# Autodesk Inventor assembly: FEM-Träger-Baugruppe1
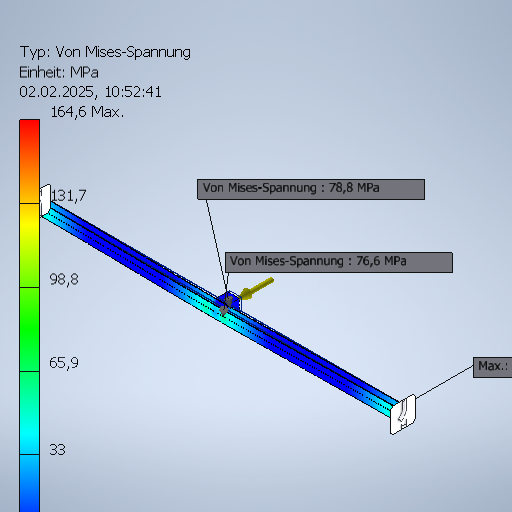
[picture p0: Inventor's stored thumbnail of the model, 512x512]
Saved by Autodesk Inventor 2025 (Build 290162010, 162A)
## iProperties
Created: 2025-02-02
Part Number: FEM-Träger-Baugruppe1
Document SubType Name: Assembly
Designer: Admin
Mass: 428.356 g
Surface Area: 1663.33 cm^2
Volume: 158.65 cm^3
Density: 2.7 g/cm^3
Author: Admin
## Documents named in this file (9)
- C:\Users\Admin\GIT\HDVKBM\CAD\Krandemonstrator\FEM-Träger-Baugruppe1.iam
- C:\Users\Admin\GIT\HDVKBM\CAD\Krandemonstrator\Träger.ipt
- C:\Users\Admin\GIT\HDVKBM\CAD\Krandemonstrator\Belastungsfläche.ipt
- C:\Users\Admin\GIT\HDVKBM\CAD\Krandemonstrator\FEM-Träger-Baugruppe1\AIP\FEA\eym8wc95s.fins
- C:\Users\Admin\GIT\HDVKBM\CAD\Krandemonstrator\FEM-Träger-Baugruppe1\AIP\FEA\eym8wc95s.fsat
- C:\Users\Admin\GIT\HDVKBM\CAD\Krandemonstrator\FEM-Träger-Baugruppe1\AIP\FEA\eym8wc95s.ftes
- C:\Users\Admin\GIT\HDVKBM\CAD\Krandemonstrator\FEM-Träger-Baugruppe1\AIP\FEA\eym8wc95s.fwiz
- C:\Users\Admin\GIT\HDVKBM\CAD\Krandemonstrator\FEM-Träger-Baugruppe1\AIP\FEA\eym8wc97k.fmsh
- C:\Users\Admin\GIT\HDVKBM\CAD\Krandemonstrator\FEM-Träger-Baugruppe1\AIP\FEA\eym8wc97l.fres
## Components (2 placed, 2 different names)
1. Träger:1 — Verschiebbar:1
2. Belastungsfläche:1 — Verschiebbar:1
## Relationships (1: TranslationJoint 1)
- Verschiebbar:1 [TranslationJoint]: Träger:1 ↔ Belastungsfläche:1
## Named parameters: sa_0 = 50000
note: some values were not read from the file. Shown as the stored number, unit unknown: "sa_0".
